# Autodesk Inventor assembly: MVPV1
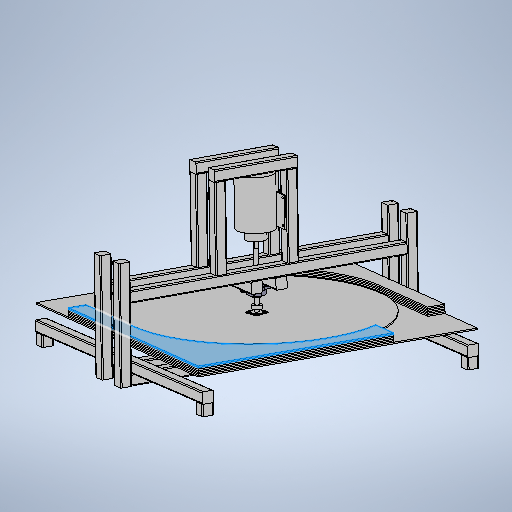
[picture p0: Inventor's stored thumbnail of the model, 512x512]
Saved by Autodesk Inventor 2025.1 (Build 291241000, 241)
## iProperties
Created: 2025-10-12
Part Number: MVPV1
Document SubType Name: Assembly
Designer: jonas
Author: jonas
## Documents named in this file (16)
- C:\Users\jonas\Documents\Studium\Master\3.Semester\StudentProject\SpinLauncher\drawings\MVPV2.iam
- C:\Users\jonas\Documents\Studium\Master\3.Semester\StudentProject\SpinLauncher\drawings\Item4040MotorVerticalV1.ipt
- C:\Users\jonas\Documents\Studium\Master\3.Semester\StudentProject\SpinLauncher\drawings\Item4040MotorHorizontalV1.ipt
- C:\Users\jonas\Documents\Studium\Master\3.Semester\StudentProject\SpinLauncher\drawings\Item4040RotorHorizontalV1.ipt
- C:\Users\jonas\Documents\Studium\Master\3.Semester\StudentProject\SpinLauncher\drawings\Item4040RotorVerticalV1.ipt
- C:\Users\jonas\Documents\Studium\Master\3.Semester\StudentProject\SpinLauncher\drawings\FlanschV1.ipt
- C:\Users\jonas\Documents\Studium\Master\3.Semester\StudentProject\SpinLauncher\drawings\RotorDiskV1.ipt
- C:\Users\jonas\Documents\Studium\Master\3.Semester\StudentProject\SpinLauncher\drawings\FlanschKugellager15mm\7508860.iam
- C:\Users\jonas\Documents\Studium\Master\3.Semester\StudentProject\SpinLauncher\drawings\Item4040BearingHolder.ipt
- C:\Users\jonas\Documents\Studium\Master\3.Semester\StudentProject\SpinLauncher\drawings\ShaftNut300mmV1.ipt
- C:\Users\jonas\Documents\Studium\Master\3.Semester\StudentProject\SpinLauncher\drawings\ShaftManschette15mmV1.ipt
- C:\Users\jonas\Documents\Studium\Master\3.Semester\StudentProject\SpinLauncher\drawings\MotorV2.ipt
- C:\Users\jonas\Documents\Studium\Master\3.Semester\StudentProject\SpinLauncher\drawings\StatorGroundPlateV1.ipt
- C:\Users\jonas\Documents\Studium\Master\3.Semester\StudentProject\SpinLauncher\drawings\BoundaryV1.ipt
- C:\Users\jonas\Documents\Studium\Master\3.Semester\StudentProject\SpinLauncher\drawings\Item4040RotorHorizontalStabilityV1.ipt
- C:\Users\jonas\Documents\Studium\Master\3.Semester\StudentProject\SpinLauncher\drawings\Item4040RotorVerticalStabilityHolderV1.ipt
## Components (45 placed, 15 different names)
1. Item4040MotorVerticalV1:1 — Flush:5, Mate:4, Flush:6, Mate:8, Flush:13, Mate:39, Flush:32
2. Item4040MotorVerticalV1:2 — Mate:3, Flush:3, Flush:4, Mate:7, Flush:11, Mate:40, Flush:33
3. Item4040MotorHorizontalV1:1 — Flush:5, Mate:4, Flush:6, Mate:6, Flush:9, Flush:10, Flush:26
4. Item4040MotorHorizontalV1:2 — Mate:3, Flush:3, Flush:4, Mate:5, Flush:7, Flush:8, Flush:26
5. Item4040MotorVerticalV1:3 — Mate:6, Flush:9, Flush:10, Flush:14
6. Item4040MotorVerticalV1:4 — Mate:5, Flush:7, Flush:8, Flush:12
7. Item4040RotorHorizontalV1:1 — Mate:7, Flush:11, Flush:12, Mate:9, Mate:11, Flush:15, Flush:17, Mate:21, Flush:29, Flush:30
8. Item4040RotorHorizontalV1:2 — Mate:8, Flush:13, Flush:14, Mate:10, Mate:12, Flush:16, Flush:18, Mate:22, Mate:82
9. Item4040RotorHorizontalV1:3 — Mate:14, Flush:19, Flush:22, Flush:24, Mate:73, Mate:74, Mate:78, Mate:80
10. Item4040RotorHorizontalV1:4 — Mate:13, Flush:20, Flush:21, Flush:23, Flush:47, Flush:48
11. Item4040RotorVerticalV1:1 — Mate:10, Flush:18, Flush:24, Mate:81
12. Item4040RotorVerticalV1:2 — Mate:9, Flush:17, Flush:23, Flush:50
13. Item4040RotorVerticalV1:3 — Mate:12, Flush:16, Mate:14, Flush:19, Flush:22, Flush:25, Flush:27, Mate:79
14. Item4040RotorVerticalV1:4 — Mate:11, Flush:15, Mate:13, Flush:20, Flush:21, Flush:25, Flush:27
15. FlanschV1:1 — Mate:15, Mate:16, Flush:31, Mate:35, Mate:44
16. RotorDiskV1:1 — Mate:15, Mate:16, Mate:76, Mate:77
17. Item4040BearingHolder:2 — Mate:22, Flush:30, Mate:26, Mate:27
18. Item4040BearingHolder:3 — Mate:21, Flush:29, Mate:23, Mate:25, Mate:26
19. 7508860:2 [sub-assembly] — Mate:23, Mate:25, Mate:27, Mate:42
20. ShaftNut300mmV1:1 — Flush:31, Mate:33, Mate:34, Mate:38, Mate:41, Mate:42, Mate:44, Mate:45, Mate:47, Mate:75
21. ShaftManschette15mmV1:1 — Mate:33, Mate:35
22. ShaftManschette15mmV1:2 — Mate:34, Mate:76
23. MotorV2:1 — Mate:38, Mate:39, Mate:40, Mate:41, Flush:32, Flush:33, Mate:82
24. StatorGroundPlateV1:1 — Mate:45, Mate:46, Flush:34, Mate:53, Mate:54, Mate:55, Mate:56, Mate:57, Mate:63, Flush:46, Mate:64, Mate:65, Mate:66, Mate:67, Mate:68, Mate:77
25. BoundaryV1:1 — Mate:46, Mate:47, Flush:34, Mate:48, Flush:35
26. BoundaryV1:2 — Mate:48, Mate:49, Flush:35, Mate:53, Flush:36
27. BoundaryV1:3 — Mate:49, Mate:50, Mate:54, Flush:36, Flush:37
28. BoundaryV1:4 — Mate:50, Mate:51, Mate:57, Flush:37, Flush:38
29. BoundaryV1:5 — Mate:51, Mate:52, Mate:56, Flush:38, Flush:39
30. BoundaryV1:12 — Mate:52, Mate:55, Flush:39
31. BoundaryV1:13 — Mate:63, Flush:45, Flush:46, Mate:64
32. BoundaryV1:14 — Flush:45
33. BoundaryV1:15 — Mate:65
34. BoundaryV1:16 — Mate:66
35. BoundaryV1:17 — Mate:67
36. BoundaryV1:18 — Mate:68
37. Item4040BearingHolder:4 — Mate:73, Flush:48
38. Item4040BearingHolder:5 — Mate:74, Flush:47
39. 7508860:3 [sub-assembly] — Mate:75
40. Item4040RotorHorizontalStabilityV1:1 — Mate:80, Mate:81, Flush:49, Flush:50, Mate:83, Flush:51, Flush:52, Mate:84, Flush:53, Flush:54
41. Item4040RotorHorizontalStabilityV1:2 — Mate:78, Mate:79, Flush:49, Mate:85, Flush:55, Flush:56, Mate:86, Flush:57, Flush:58
42. Item4040RotorVerticalStabilityHolderV1:1 — Mate:83, Flush:51, Flush:52
43. Item4040RotorVerticalStabilityHolderV1:2 — Mate:85, Flush:55, Flush:56
44. Item4040RotorVerticalStabilityHolderV1:3 — Mate:86, Flush:57, Flush:58
45. Item4040RotorVerticalStabilityHolderV1:4 — Mate:84, Flush:53, Flush:54
## Relationships (126: Mate 71, Flush 55)
- Mate:3: Item4040MotorVerticalV1:2 ↔ Item4040MotorHorizontalV1:2
- Flush:3: Item4040MotorVerticalV1:2 ↔ Item4040MotorHorizontalV1:2
- Flush:4: Item4040MotorVerticalV1:2 ↔ Item4040MotorHorizontalV1:2
- Flush:5: Item4040MotorVerticalV1:1 ↔ Item4040MotorHorizontalV1:1
- Mate:4: Item4040MotorVerticalV1:1 ↔ Item4040MotorHorizontalV1:1
- Flush:6: Item4040MotorVerticalV1:1 ↔ Item4040MotorHorizontalV1:1
- Mate:5: Item4040MotorHorizontalV1:2 ↔ Item4040MotorVerticalV1:4
- Flush:7: Item4040MotorHorizontalV1:2 ↔ Item4040MotorVerticalV1:4
- Flush:8: Item4040MotorHorizontalV1:2 ↔ Item4040MotorVerticalV1:4
- Mate:6: Item4040MotorHorizontalV1:1 ↔ Item4040MotorVerticalV1:3
- Flush:9: Item4040MotorHorizontalV1:1 ↔ Item4040MotorVerticalV1:3
- Flush:10: Item4040MotorHorizontalV1:1 ↔ Item4040MotorVerticalV1:3
- Mate:7: Item4040MotorVerticalV1:2 ↔ Item4040RotorHorizontalV1:1
- Flush:11: Item4040MotorVerticalV1:2 ↔ Item4040RotorHorizontalV1:1
- Flush:12: Item4040MotorVerticalV1:4 ↔ Item4040RotorHorizontalV1:1
- Mate:8: Item4040MotorVerticalV1:1 ↔ Item4040RotorHorizontalV1:2
- Flush:13: Item4040MotorVerticalV1:1 ↔ Item4040RotorHorizontalV1:2
- Flush:14: Item4040MotorVerticalV1:3 ↔ Item4040RotorHorizontalV1:2
- Mate:9: Item4040RotorHorizontalV1:1 ↔ Item4040RotorVerticalV1:2
- Mate:10: Item4040RotorHorizontalV1:2 ↔ Item4040RotorVerticalV1:1
- Mate:11: Item4040RotorHorizontalV1:1 ↔ Item4040RotorVerticalV1:4
- Mate:12: Item4040RotorHorizontalV1:2 ↔ Item4040RotorVerticalV1:3
- Flush:15: Item4040RotorHorizontalV1:1 ↔ Item4040RotorVerticalV1:4
- Flush:16: Item4040RotorHorizontalV1:2 ↔ Item4040RotorVerticalV1:3
- Flush:17: Item4040RotorHorizontalV1:1 ↔ Item4040RotorVerticalV1:2
- Flush:18: Item4040RotorHorizontalV1:2 ↔ Item4040RotorVerticalV1:1
- Mate:13: Item4040RotorHorizontalV1:4 ↔ Item4040RotorVerticalV1:4
- Mate:14: Item4040RotorHorizontalV1:3 ↔ Item4040RotorVerticalV1:3
- Flush:19: Item4040RotorHorizontalV1:3 ↔ Item4040RotorVerticalV1:3
- Flush:20: Item4040RotorHorizontalV1:4 ↔ Item4040RotorVerticalV1:4
- Flush:21: Item4040RotorHorizontalV1:4 ↔ Item4040RotorVerticalV1:4
- Flush:22: Item4040RotorHorizontalV1:3 ↔ Item4040RotorVerticalV1:3
- Flush:23: Item4040RotorHorizontalV1:4 ↔ Item4040RotorVerticalV1:2
- Flush:24: Item4040RotorHorizontalV1:3 ↔ Item4040RotorVerticalV1:1
- Flush:25: Item4040RotorVerticalV1:3 ↔ Item4040RotorVerticalV1:4
- Flush:26: Item4040MotorHorizontalV1:1 ↔ Item4040MotorHorizontalV1:2
- Flush:27: Item4040RotorVerticalV1:3 ↔ Item4040RotorVerticalV1:4
- Mate:15: FlanschV1:1 ↔ RotorDiskV1:1
- Mate:16: FlanschV1:1 ↔ RotorDiskV1:1
- Mate:21: Item4040RotorHorizontalV1:1 ↔ Item4040BearingHolder:3
- Mate:22: Item4040RotorHorizontalV1:2 ↔ Item4040BearingHolder:2
- Flush:29: Item4040RotorHorizontalV1:1 ↔ Item4040BearingHolder:3
- Flush:30: Item4040RotorHorizontalV1:1 ↔ Item4040BearingHolder:2
- Mate:23: Item4040BearingHolder:3 ↔ 7508860:2
- Mate:25 (-20 mm): Item4040BearingHolder:3 ↔ 7508860:2
- Mate:26 (-130 mm): Item4040BearingHolder:2 ↔ Item4040BearingHolder:3
- Mate:27 (-20 mm): Item4040BearingHolder:2 ↔ 7508860:2
- Flush:31: FlanschV1:1 ↔ ShaftNut300mmV1:1
- Mate:33: ShaftNut300mmV1:1 ↔ ShaftManschette15mmV1:1
- Mate:34: ShaftNut300mmV1:1 ↔ ShaftManschette15mmV1:2
- Mate:35 (10 mm): FlanschV1:1 ↔ ShaftManschette15mmV1:1
- Mate:38: ShaftNut300mmV1:1 ↔ MotorV2:1
- Mate:39: Item4040MotorVerticalV1:1 ↔ MotorV2:1
- Mate:40: Item4040MotorVerticalV1:2 ↔ MotorV2:1
- Mate:41: ShaftNut300mmV1:1 ↔ MotorV2:1
- Flush:32 (8.75 mm): Item4040MotorVerticalV1:1 ↔ MotorV2:1
- Flush:33 (-8.75 mm): Item4040MotorVerticalV1:2 ↔ MotorV2:1
- Mate:42: 7508860:2 ↔ ShaftNut300mmV1:1
- Mate:44: FlanschV1:1 ↔ ShaftNut300mmV1:1
- Mate:45: ShaftNut300mmV1:1 ↔ StatorGroundPlateV1:1
- Mate:46: StatorGroundPlateV1:1 ↔ BoundaryV1:1
- Mate:47: ShaftNut300mmV1:1 ↔ BoundaryV1:1
- Flush:34: StatorGroundPlateV1:1 ↔ BoundaryV1:1
- Mate:48: BoundaryV1:1 ↔ BoundaryV1:2
- Mate:49: BoundaryV1:2 ↔ BoundaryV1:3
- Mate:50: BoundaryV1:3 ↔ BoundaryV1:4
- Mate:51: BoundaryV1:4 ↔ BoundaryV1:5
- Mate:52: BoundaryV1:5 ↔ BoundaryV1:12
- Flush:35: BoundaryV1:1 ↔ BoundaryV1:2
- Mate:53: StatorGroundPlateV1:1 ↔ BoundaryV1:2
- Mate:54: StatorGroundPlateV1:1 ↔ BoundaryV1:3
- Mate:55: StatorGroundPlateV1:1 ↔ BoundaryV1:12
- Mate:56: StatorGroundPlateV1:1 ↔ BoundaryV1:5
- Mate:57: StatorGroundPlateV1:1 ↔ BoundaryV1:4
- Flush:36: BoundaryV1:2 ↔ BoundaryV1:3
- Flush:37: BoundaryV1:3 ↔ BoundaryV1:4
- Flush:38: BoundaryV1:4 ↔ BoundaryV1:5
- Flush:39: BoundaryV1:5 ↔ BoundaryV1:12
- [Mate]: BoundaryV1:13 ↔ BoundaryV1:14
- [Mate]: BoundaryV1:14 ↔ BoundaryV1:15
- [Mate]: BoundaryV1:15 ↔ BoundaryV1:16
- [Mate]: BoundaryV1:16 ↔ BoundaryV1:17
- [Mate]: BoundaryV1:17 ↔ BoundaryV1:18
- [Flush]: BoundaryV1:13 ↔ BoundaryV1:14
- [Flush]: BoundaryV1:14 ↔ BoundaryV1:15
- [Flush]: BoundaryV1:15 ↔ BoundaryV1:16
- [Flush]: BoundaryV1:16 ↔ BoundaryV1:17
- [Flush]: BoundaryV1:17 ↔ BoundaryV1:18
- Mate:63: StatorGroundPlateV1:1 ↔ BoundaryV1:13
- Flush:45: BoundaryV1:13 ↔ BoundaryV1:14
- Flush:46: StatorGroundPlateV1:1 ↔ BoundaryV1:13
- Mate:64: StatorGroundPlateV1:1 ↔ BoundaryV1:13
- Mate:65: StatorGroundPlateV1:1 ↔ BoundaryV1:15
- Mate:66: StatorGroundPlateV1:1 ↔ BoundaryV1:16
- Mate:67: StatorGroundPlateV1:1 ↔ BoundaryV1:17
- Mate:68: StatorGroundPlateV1:1 ↔ BoundaryV1:18
- [Mate]: Item4040BearingHolder:5 ↔ 7508860:3
- [Mate] (-20 mm): Item4040BearingHolder:5 ↔ 7508860:3
- [Mate] (-130 mm): Item4040BearingHolder:4 ↔ Item4040BearingHolder:5
- [Mate] (-20 mm): Item4040BearingHolder:4 ↔ 7508860:3
- Mate:73: Item4040RotorHorizontalV1:3 ↔ Item4040BearingHolder:4
- Mate:74: Item4040RotorHorizontalV1:3 ↔ Item4040BearingHolder:5
- Flush:47: Item4040RotorHorizontalV1:4 ↔ Item4040BearingHolder:5
- Flush:48: Item4040RotorHorizontalV1:4 ↔ Item4040BearingHolder:4
- Mate:75: ShaftNut300mmV1:1 ↔ 7508860:3
- Mate:76: RotorDiskV1:1 ↔ ShaftManschette15mmV1:2
- Mate:77 (3 mm): RotorDiskV1:1 ↔ StatorGroundPlateV1:1
- Mate:78: Item4040RotorHorizontalV1:3 ↔ Item4040RotorHorizontalStabilityV1:2
- Mate:79: Item4040RotorVerticalV1:3 ↔ Item4040RotorHorizontalStabilityV1:2
- Mate:80: Item4040RotorHorizontalV1:3 ↔ Item4040RotorHorizontalStabilityV1:1
- Mate:81: Item4040RotorVerticalV1:1 ↔ Item4040RotorHorizontalStabilityV1:1
- Flush:49: Item4040RotorHorizontalStabilityV1:1 ↔ Item4040RotorHorizontalStabilityV1:2
- Flush:50 (-423.75 mm): Item4040RotorVerticalV1:2 ↔ Item4040RotorHorizontalStabilityV1:1
- Mate:82 (-500 mm): Item4040RotorHorizontalV1:2 ↔ MotorV2:1
- Mate:83: Item4040RotorHorizontalStabilityV1:1 ↔ Item4040RotorVerticalStabilityHolderV1:1
- Flush:51: Item4040RotorHorizontalStabilityV1:1 ↔ Item4040RotorVerticalStabilityHolderV1:1
- Flush:52: Item4040RotorHorizontalStabilityV1:1 ↔ Item4040RotorVerticalStabilityHolderV1:1
- Mate:84: Item4040RotorHorizontalStabilityV1:1 ↔ Item4040RotorVerticalStabilityHolderV1:4
- Flush:53: Item4040RotorHorizontalStabilityV1:1 ↔ Item4040RotorVerticalStabilityHolderV1:4
- Flush:54: Item4040RotorHorizontalStabilityV1:1 ↔ Item4040RotorVerticalStabilityHolderV1:4
- Mate:85: Item4040RotorHorizontalStabilityV1:2 ↔ Item4040RotorVerticalStabilityHolderV1:2
- Flush:55: Item4040RotorHorizontalStabilityV1:2 ↔ Item4040RotorVerticalStabilityHolderV1:2
- Flush:56: Item4040RotorHorizontalStabilityV1:2 ↔ Item4040RotorVerticalStabilityHolderV1:2
- Mate:86: Item4040RotorHorizontalStabilityV1:2 ↔ Item4040RotorVerticalStabilityHolderV1:3
- Flush:57: Item4040RotorHorizontalStabilityV1:2 ↔ Item4040RotorVerticalStabilityHolderV1:3
- Flush:58: Item4040RotorHorizontalStabilityV1:2 ↔ Item4040RotorVerticalStabilityHolderV1:3
## Named parameters: d99_d84 = 0 mm, d100_d85 = 0 mm, d101_d86 = 0 mm, d102_d87 = 0 mm, d103_d88 = 0 mm, d104_d89 = 0 mm, d105_d95 = 0 mm, d106_d96 = 0 mm, d107_d97 = 0 mm, d108_d98 = 0 mm, d117_d52 = 0 mm, d118_d54 = -20 mm, d119_d56 = -130 mm, d120_d57 = -20 mm
